# Autodesk Inventor assembly: gripper
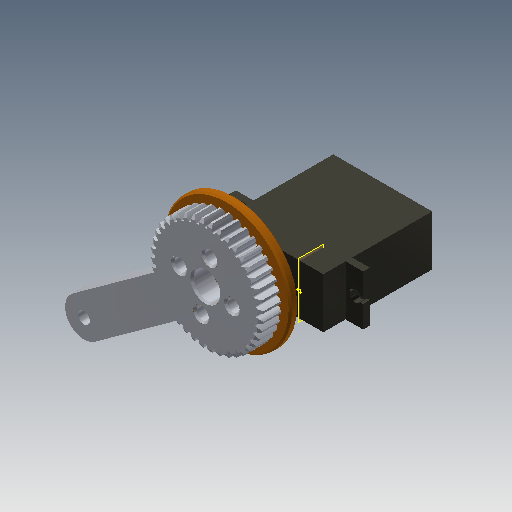
[picture p0: Inventor's stored thumbnail of the model, 512x512]
Saved by Autodesk Inventor 2018 (Build 220112000, 112)
## iProperties
Created: 2020-01-19
Part Number: gripper
Document SubType Name: Assembly
Designer: anirudh
Author: anirudh
## Documents named in this file (4)
- D:\Silicon Sharks\2019-2020\Gripper\gripper.iam
- D:\Silicon Sharks\2019-2020\Gripper\gripperServo.ipt
- D:\Silicon Sharks\2019-2020\Gripper\REV-41-1363.ipt
- D:\Silicon Sharks\2019-2020\Gripper\gripperPart1.ipt
## Components (3 placed, 3 different names)
1. gripperServo:1 — Mate:1, Mate:2
2. REV-41-1363:1 — Mate:1, Mate:2, Mate:3, Mate:4, Mate:5
3. gripperPart1:1 — Mate:3, Mate:4, Mate:5
## Relationships (5: Mate 5)
- Mate:1: gripperServo:1 ↔ REV-41-1363:1
- Mate:2: gripperServo:1 ↔ REV-41-1363:1
- Mate:3: REV-41-1363:1 ↔ gripperPart1:1
- Mate:4: REV-41-1363:1 ↔ gripperPart1:1
- Mate:5: REV-41-1363:1 ↔ gripperPart1:1
